# Autodesk Inventor assembly: Assembly1
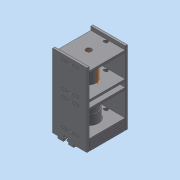
[picture p0: Inventor's stored thumbnail of the model, 180x180]
Saved by Autodesk Inventor 2016 SP1 (Build 200210100, 210)
## iProperties
Created: 2016-03-20
Part Number: Assembly1
Document SubType Name: Assembly
Designer: Mohamed A.
Author: Mohamed A.
## Documents named in this file (12)
- C:\Users\Mohamed\Documents\inventor\Faboscope\Camera\new\Assembly1.iam
- C:\Users\Mohamed\Documents\inventor\Faboscope\Camera\new\Board.ipt
- C:\Users\Mohamed\Documents\inventor\Faboscope\Camera\new\Part2.ipt
- C:\Users\Mohamed\Documents\inventor\Faboscope\Lenses\Eye-Piece.ipt
- C:\Users\Mohamed\Documents\inventor\Faboscope\Camera\new\Part4.ipt
- C:\Users\Mohamed\Documents\inventor\Faboscope\Camera\new\Part3.ipt
- C:\Users\Mohamed\Documents\inventor\Faboscope\Laser Cut\Camera-Holder\Camera-Holder_Mount-Bottom.ipt
- C:\Users\Mohamed\Documents\inventor\Faboscope\Lenses\Objective-Lens.ipt
- C:\Users\Mohamed\Documents\inventor\Faboscope\Camera\new\Part5.ipt
- C:\Users\Mohamed\Documents\inventor\Faboscope\Camera\new\Part6.ipt
- C:\Users\Mohamed\Documents\inventor\Faboscope\Camera\new\Part7.ipt
- C:\Users\Mohamed\Documents\inventor\Faboscope\Camera\new\Part8.ipt
## Components (13 placed, 11 different names)
1. Board:1 — Mate:1
2. Part2:1
3. Part2:2
4. Eye-Piece:1 — Mate:1, Mate:2, Mate:3, Mate:4, Flush:1
5. Part4:1 — Mate:2
6. Part3:1
7. Camera-Holder_Mount-Bottom:1
8. Objective-Lens:1 — Mate:3, Mate:4, Flush:2, Flush:3, Angle:1
9. Part6:1 — Flush:2
10. Part7:1 — Flush:3, Flush:4, Mate:5, Mate:6, Flush:7
11. Part5:1 — Flush:1
12. Part8:1 — Flush:4, Mate:5, Mate:6, Flush:5, Flush:6
13. Part8:2 — Flush:5, Flush:6, Flush:7
## Relationships (14: Flush 7, Mate 6, Angle 1)
- Mate:1: Board:1 ↔ Eye-Piece:1
- Mate:2: Eye-Piece:1 ↔ Part4:1
- Mate:3: Eye-Piece:1 ↔ Objective-Lens:1
- Mate:4 (-46.2 mm): Eye-Piece:1 ↔ Objective-Lens:1
- Flush:1: Eye-Piece:1 ↔ Part5:1
- Flush:2: Objective-Lens:1 ↔ Part6:1
- Flush:3: Objective-Lens:1 ↔ Part7:1
- Flush:4: Part7:1 ↔ Part8:1
- Mate:5: Part7:1 ↔ Part8:1
- Mate:6: Part7:1 ↔ Part8:1
- Flush:5: Part8:1 ↔ Part8:2
- Flush:6: Part8:1 ↔ Part8:2
- Flush:7: Part7:1 ↔ Part8:2
- Angle:1 (0 deg): Objective-Lens:1
